# Autodesk Inventor assembly: Side Solar Panel
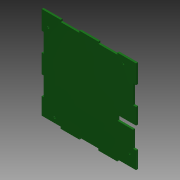
[picture p0: Inventor's stored thumbnail of the model, 180x180]
Saved by Autodesk Inventor 2015 SP1 (Build 190203100, 203)
## iProperties
Created: 2015-10-18
Part Number: Side Solar Panel
Document SubType Name: Assembly
Designer: Kartikye
Author: Kartikye
## Documents named in this file (3)
- C:\Users\Kartikye\Documents\GitHub\SASSat\Structure\V5\Side Solar Panel with Switch.iam
- C:\Users\Kartikye\Documents\GitHub\SASSat\Structure\Solar Cell.ipt
- C:\Users\Kartikye\Documents\GitHub\SASSat\Structure\V5\Side Panel with Switch.ipt
## Components (9 placed, 2 different names)
1. Side Panel with Switch:1 — Mate:1, Flush:1, Mate:2, Mate:3, Flush:2, Mate:4, Mate:5, Mate:6, Flush:3, Flush:4, Mate:7, Mate:8, Mate:9, Flush:5, Mate:10, Mate:11, Flush:6, Mate:12, Mate:13, Flush:7, Flush:8, Mate:14, Mate:15, Mate:16
2. Solar Cell:1 — Mate:1, Flush:1, Mate:2
3. Solar Cell:2 — Mate:13, Flush:7, Flush:8
4. Solar Cell:3 — Mate:11, Flush:6, Mate:12
5. Solar Cell:4 — Mate:9, Flush:5, Mate:10
6. Solar Cell:5 — Mate:6, Flush:3, Flush:4
7. Solar Cell:6 — Mate:5, Mate:7, Mate:8
8. Solar Cell:7 — Mate:3, Flush:2, Mate:4
9. Solar Cell:8 — Mate:14, Mate:15, Mate:16
## Relationships (24: Mate 16, Flush 8)
- Mate:1: Side Panel with Switch:1 ↔ Solar Cell:1
- Flush:1 (-2 mm): Side Panel with Switch:1 ↔ Solar Cell:1
- Mate:2 (-28.4 mm): Side Panel with Switch:1 ↔ Solar Cell:1
- Mate:3: Side Panel with Switch:1 ↔ Solar Cell:7
- Flush:2 (1.4 mm): Side Panel with Switch:1 ↔ Solar Cell:7
- Mate:4 (-19.2 mm): Side Panel with Switch:1 ↔ Solar Cell:7
- Mate:5: Side Panel with Switch:1 ↔ Solar Cell:6
- Mate:6: Side Panel with Switch:1 ↔ Solar Cell:5
- Flush:3 (2 mm): Side Panel with Switch:1 ↔ Solar Cell:5
- Flush:4 (31.4 mm): Side Panel with Switch:1 ↔ Solar Cell:5
- Mate:7 (-28.5 mm): Side Panel with Switch:1 ↔ Solar Cell:6
- Mate:8 (-48.6 mm): Side Panel with Switch:1 ↔ Solar Cell:6
- Mate:9: Side Panel with Switch:1 ↔ Solar Cell:4
- Flush:5 (31.4 mm): Side Panel with Switch:1 ↔ Solar Cell:4
- Mate:10 (-48.6 mm): Side Panel with Switch:1 ↔ Solar Cell:4
- Mate:11: Side Panel with Switch:1 ↔ Solar Cell:3
- Flush:6 (21.5 mm): Side Panel with Switch:1 ↔ Solar Cell:3
- Mate:12 (-48.4 mm): Side Panel with Switch:1 ↔ Solar Cell:3
- Mate:13: Side Panel with Switch:1 ↔ Solar Cell:2
- Flush:7 (21.3 mm): Side Panel with Switch:1 ↔ Solar Cell:2
- Flush:8 (1.4 mm): Side Panel with Switch:1 ↔ Solar Cell:2
- Mate:14: Side Panel with Switch:1 ↔ Solar Cell:8
- Mate:15 (-48.4 mm): Side Panel with Switch:1 ↔ Solar Cell:8
- Mate:16 (-18.6 mm): Side Panel with Switch:1 ↔ Solar Cell:8
